# Autodesk Inventor assembly: rendering_aslm_assembly
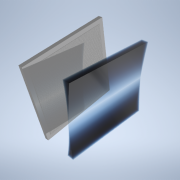
[picture p0: Inventor's stored thumbnail of the model, 180x180]
Saved by Autodesk Inventor 2021 (Build 250183000, 183)
## iProperties
Created: 2021-06-18
Part Number: rendering_aslm_assembly
Document SubType Name: Assembly
Designer: MicroscopyInnovation
Author: MicroscopyInnovation
## Documents named in this file (3)
- C:\Users\MicroscopyInnovation\Documents\Inventor\NatProtocolsManuscript\rendering_aslm_assembly_2.iam
- C:\Users\MicroscopyInnovation\Documents\Inventor\NatProtocolsManuscript\rendering_light_sheet.ipt
- C:\Users\MicroscopyInnovation\Documents\Inventor\NatProtocolsManuscript\rendering_cmos_chip.ipt
## Components (2 placed, 2 different names)
1. rendering_light_sheet:1 — Angle:1
2. rendering_cmos_chip:1 — Angle:1
## Relationships (1: Angle 1)
- Angle:1 (10 deg): rendering_light_sheet:1 ↔ rendering_cmos_chip:1
